# Autodesk Inventor assembly: Drawdio
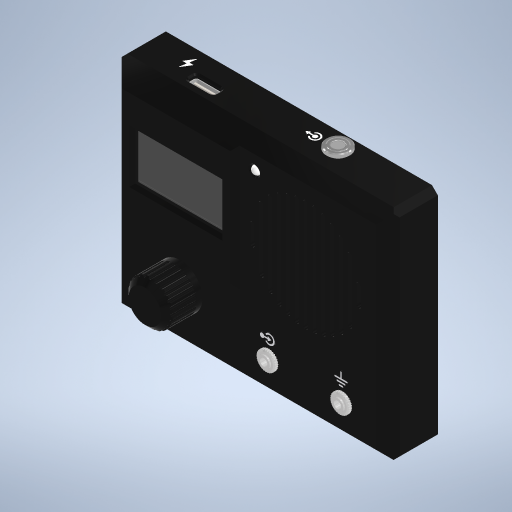
[picture p0: Inventor's stored thumbnail of the model, 512x512]
Saved by Autodesk Inventor 2024 (Build 280153000, 153)
## iProperties
Created: 2025-09-12
Part Number: Drawdio
Document SubType Name: Assembly
Designer: Login
Author: Login
## Documents named in this file (13)
- D:\Inventor\Projects\Drawdio\Drawdio.iam
- D:\Inventor\Projects\Components\Speaker 40mm.ipt
- D:\Inventor\Projects\Drawdio\Drawdio_BOT.ipt
- D:\Inventor\Projects\Drawdio\Drawdio_TOP.ipt
- D:\Inventor\Projects\Drawdio\2.5mm jack.ipt
- D:\Inventor\Projects\Drawdio\3mm LED.ipt
- D:\Inventor\Projects\Drawdio\Encder Knob.ipt
- D:\Inventor\Projects\Nixie analizator v2.0\import\101-CONN-3.5mm Stereo Connector.ipt
- D:\Inventor\Projects\Drawdio\Import\2.5mm jack nut.ipt
- D:\Inventor\Projects\Fasteners\DIN-7985 M2 Phillips Head Screw\DIN-7985_M2x6.ipt
- D:\Inventor\Projects\Fasteners\DIN-934 Nut\DIN-934_Nut_M2.ipt
- D:\Inventor\Projects\Fasteners\DIN-7985 M2 Phillips Head Screw\DIN-7985_M2x8.ipt
- D:\Inventor\Projects\Drawdio\Import\Altium\Drawdio_Step_Rev.1.2._2025-09-14\Drawdio_Step_Rev.1.2._2025-09-14.ipt
## Components (25 placed, 12 different names)
1. Drawdio_BOT:1 — Mate:10, Mate:11, Mate:12, Mate:13, Mate:14, Insert:15, Insert:16, Insert:18, Insert:19, Insert:29, Angle:7, Insert:34, Insert:35, Insert:36, Insert:37, Insert:38, Insert:40, Insert:41, Insert:42, Insert:43
2. Drawdio_TOP:1 — Mate:11, Mate:12, Mate:13, Mate:14, Mate:15, Mate:16, Angle:1, Angle:2, Angle:3, Insert:3, Angle:5, Insert:4, Insert:5, Mate:22, Mate:23, Insert:6, Angle:6, Insert:7, Insert:8, Insert:30, Insert:31, Insert:32, Insert:33, Angle:8, Angle:9, Angle:10, Angle:11
3. Encder Knob:1 — Insert:44, Mate:24
4. Drawdio_Step_Rev.1.2._2025-09-14:1 — Insert:38, Insert:39, Insert:40, Insert:41, Insert:42, Insert:43, Insert:44, Mate:24
5. Speaker 40mm:1 — Mate:15, Mate:16, Angle:1
6. 2.5mm jack:1 — Angle:3, Insert:4
7. 2.5mm jack:2 — Angle:2, Insert:5
8. 101-CONN-3.5mm Stereo Connector:1 — Insert:6, Angle:6
9. 3mm LED:1 — Insert:3, Angle:5
10. 2.5mm jack nut:1 — Insert:7
11. 2.5mm jack nut:2 — Insert:8
12. DIN-7985_M2x6:2 — Insert:15
13. DIN-7985_M2x6:3 — Insert:16
14. DIN-7985_M2x6:5 — Insert:18
15. DIN-7985_M2x6:6 — Insert:19
16. DIN-7985_M2x6:9 — Insert:39
17. DIN-934_Nut_M2:1 — Insert:29, Angle:7
18. DIN-934_Nut_M2:2 — Insert:30, Angle:11
19. DIN-934_Nut_M2:3 — Insert:31, Angle:8
20. DIN-934_Nut_M2:4 — Insert:32, Angle:10
21. DIN-934_Nut_M2:5 — Insert:33, Angle:9
22. DIN-7985_M2x8:1 — Insert:37
23. DIN-7985_M2x8:2 — Insert:36
24. DIN-7985_M2x8:3 — Insert:34
25. DIN-7985_M2x8:4 — Insert:35
## Relationships (46: Insert 26, Mate 10, Angle 10)
- Mate:10: Drawdio_BOT:1
- Mate:11: Drawdio_BOT:1 ↔ Drawdio_TOP:1
- Mate:12: Drawdio_BOT:1 ↔ Drawdio_TOP:1
- Mate:13: Drawdio_BOT:1 ↔ Drawdio_TOP:1
- Mate:14: Drawdio_BOT:1 ↔ Drawdio_TOP:1
- Mate:15: Drawdio_TOP:1 ↔ Speaker 40mm:1
- Mate:16: Drawdio_TOP:1 ↔ Speaker 40mm:1
- Angle:1 (-90 deg): Drawdio_TOP:1 ↔ Speaker 40mm:1
- Angle:2 (90 deg): Drawdio_TOP:1 ↔ 2.5mm jack:2
- Angle:3 (90 deg): Drawdio_TOP:1 ↔ 2.5mm jack:1
- Insert:3: Drawdio_TOP:1 ↔ 3mm LED:1
- Angle:5 (0 deg): Drawdio_TOP:1 ↔ 3mm LED:1
- Insert:4: Drawdio_TOP:1 ↔ 2.5mm jack:1
- Insert:5: Drawdio_TOP:1 ↔ 2.5mm jack:2
- Mate:22: Drawdio_TOP:1
- Mate:23: Drawdio_TOP:1
- Insert:6: Drawdio_TOP:1 ↔ 101-CONN-3.5mm Stereo Connector:1
- Angle:6 (0 deg): Drawdio_TOP:1 ↔ 101-CONN-3.5mm Stereo Connector:1
- Insert:7: Drawdio_TOP:1 ↔ 2.5mm jack nut:1
- Insert:8: Drawdio_TOP:1 ↔ 2.5mm jack nut:2
- Insert:15: Drawdio_BOT:1 ↔ DIN-7985_M2x6:2
- Insert:16: Drawdio_BOT:1 ↔ DIN-7985_M2x6:3
- Insert:18: Drawdio_BOT:1 ↔ DIN-7985_M2x6:5
- Insert:19: Drawdio_BOT:1 ↔ DIN-7985_M2x6:6
- Insert:29: Drawdio_BOT:1 ↔ DIN-934_Nut_M2:1
- Angle:7 (0 deg): Drawdio_BOT:1 ↔ DIN-934_Nut_M2:1
- Insert:30: Drawdio_TOP:1 ↔ DIN-934_Nut_M2:2
- Insert:31: Drawdio_TOP:1 ↔ DIN-934_Nut_M2:3
- Insert:32: Drawdio_TOP:1 ↔ DIN-934_Nut_M2:4
- Insert:33: Drawdio_TOP:1 ↔ DIN-934_Nut_M2:5
- Insert:34: Drawdio_BOT:1 ↔ DIN-7985_M2x8:3
- Insert:35: Drawdio_BOT:1 ↔ DIN-7985_M2x8:4
- Insert:36: Drawdio_BOT:1 ↔ DIN-7985_M2x8:2
- Insert:37: Drawdio_BOT:1 ↔ DIN-7985_M2x8:1
- Insert:38: Drawdio_BOT:1 ↔ Drawdio_Step_Rev.1.2._2025-09-14:1
- Insert:39: Drawdio_Step_Rev.1.2._2025-09-14:1 ↔ DIN-7985_M2x6:9
- Insert:40: Drawdio_BOT:1 ↔ Drawdio_Step_Rev.1.2._2025-09-14:1
- Insert:41: Drawdio_BOT:1 ↔ Drawdio_Step_Rev.1.2._2025-09-14:1
- Insert:42: Drawdio_BOT:1 ↔ Drawdio_Step_Rev.1.2._2025-09-14:1
- Insert:43: Drawdio_BOT:1 ↔ Drawdio_Step_Rev.1.2._2025-09-14:1
- Insert:44: Encder Knob:1 ↔ Drawdio_Step_Rev.1.2._2025-09-14:1
- Mate:24: Encder Knob:1 ↔ Drawdio_Step_Rev.1.2._2025-09-14:1
- Angle:8 (0 deg): Drawdio_TOP:1 ↔ DIN-934_Nut_M2:3
- Angle:9 (0 deg): Drawdio_TOP:1 ↔ DIN-934_Nut_M2:5
- Angle:10 (0 deg): Drawdio_TOP:1 ↔ DIN-934_Nut_M2:4
- Angle:11 (0 deg): Drawdio_TOP:1 ↔ DIN-934_Nut_M2:2
